# Autodesk Inventor assembly: chassis
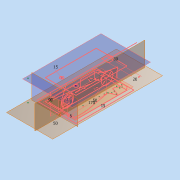
[picture p0: Inventor's stored thumbnail of the model, 180x180]
Saved by Autodesk Inventor 2022 (Build 260153000, 153)
## iProperties
Created: 2021-06-06
Part Number: chassis
Document SubType Name: Assembly
Designer: Default
Author: Default
## Documents named in this file (2)
- E:\source\repos\S21\fachübergreifend\fennec bot\fennec-jet-racer\Konstruktion\chassis.iam
- E:\source\repos\S21\fachübergreifend\fennec bot\fennec-jet-racer\Konstruktion\struktur.ipt
## Components (1 placed, 1 different names)
1. struktur:1 — Passend:1
## Relationships (1: Mate 1)
- Passend:1 [Mate]: struktur:1
